# Autodesk Inventor assembly: splitter_MIR
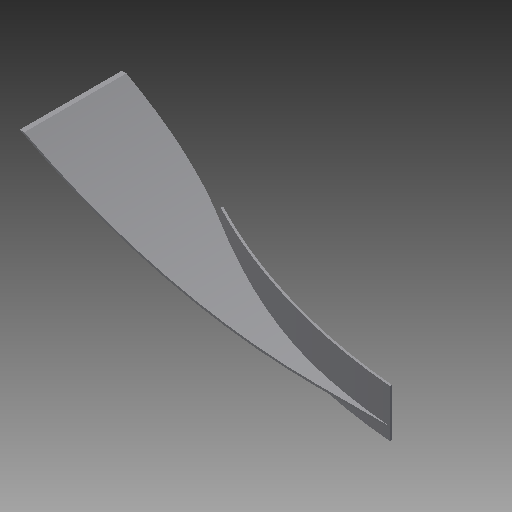
[picture p0: Inventor's stored thumbnail of the model, 512x512]
Saved by Autodesk Inventor 2018 (Build 220112000, 112)
## iProperties
Created: 2018-05-29
Part Number: splitter_MIR
Material: 一般
Document SubType Name: Assembly
Designer: ku_sk
Author: ku_sk
## Documents named in this file (3)
- D:\Users\ku_sk\Documents\Inventor\Aero\KS-15\Fr.wing\parts\splitter\splitter_MIR.iam
- D:\Users\ku_sk\Documents\Inventor\Aero\KS-15\Fr.wing\parts\splitter\parts\Part1_MIR.ipt
- D:\Users\ku_sk\Documents\Inventor\Aero\KS-15\Fr.wing\parts\splitter\parts\Part2_MIR.ipt
## Components (2 placed, 2 different names)
1. Part1_MIR:1 — メイト:3, メイト:2, メイト:1, メイト:6, メイト:5, メイト:4
2. Part2_MIR:1 — メイト:6, メイト:5, メイト:4
## Relationships (6: Mate 6)
- メイト:3 [Mate]: Part1_MIR:1
- メイト:2 [Mate]: Part1_MIR:1
- メイト:1 [Mate]: Part1_MIR:1
- メイト:6 [Mate]: Part1_MIR:1 ↔ Part2_MIR:1
- メイト:5 [Mate]: Part1_MIR:1 ↔ Part2_MIR:1
- メイト:4 [Mate]: Part1_MIR:1 ↔ Part2_MIR:1
